# Autodesk Inventor assembly: cloudcase
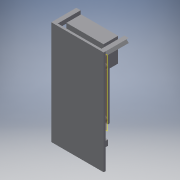
[picture p0: Inventor's stored thumbnail of the model, 180x180]
Saved by Autodesk Inventor 2018 (Build 220112000, 112)
## iProperties
Created: 2018-06-29
Part Number: cloudcase
Document SubType Name: Assembly
Designer: erwin
Author: erwin
## Documents named in this file (3)
- D:\GitHub\cloudberry-case\design\new\cloudcase.iam
- D:\GitHub\cloudberry-case\design\new\board.ipt
- D:\GitHub\cloudberry-case\design\new\bottom.ipt
## Components (2 placed, 2 different names)
1. board:1 — Flush:1, Flush:2
2. bottom:1 — Flush:1, Flush:2
## Relationships (2: Flush 2)
- Flush:1: board:1 ↔ bottom:1
- Flush:2 (3 mm): board:1 ↔ bottom:1
